# Autodesk Inventor assembly: Upperarm
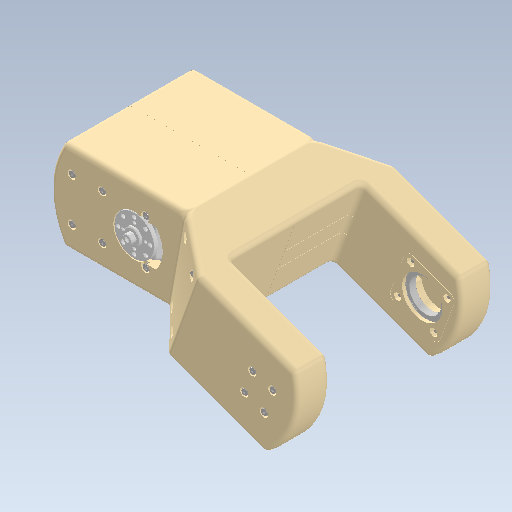
[picture p0: Inventor's stored thumbnail of the model, 512x512]
Saved by Autodesk Inventor 2021 (Build 250183000, 183)
## iProperties
Created: 2020-02-11
Part Number: Upperarm
Document SubType Name: Assembly
Designer: JochenAlt
Author: JochenAlt
## Documents named in this file (7)
- C:\Users\Jochen Alt\Documents\Daten\Projects\MiniBot\CAD\Upperarm.iam
- C:\Users\Jochen Alt\Documents\Daten\Projects\MiniBot\CAD\Upperarm.ipt
- C:\Users\Jochen Alt\Documents\Daten\Projects\MiniBot\CAD\extern\Herkulex\Herkulex DRS-040x.ipt
- C:\Users\Jochen Alt\Documents\Daten\Projects\MiniBot\CAD\extern\bearings\20x27x4\W 61704-2ZS.iam
- D:\Projects\MiniBot\CAD\extern\DIN 912\DIN 912 - M2 x 0,4 x 20 x 19.ipt
- D:\Projects\MiniBot\CAD\extern\DIN 912\DIN 912 - M2 x 0.4 x 10 x 9.ipt
- D:\Projects\MiniBot\CAD\extern\DIN 912\DIN 912 - M2 x 0,4 x 16 x 15.ipt
## Components (32 placed, 6 different names)
1. Upperarm:1 — Winkel:1, Passend:3, Fluchtend:2, Insert:1, Insert:2, Insert:3, Insert:4, Insert:5, Insert:6, Insert:7, Insert:8, Insert:9, Insert:10, Insert:11, Insert:12, Insert:13, Insert:14, Insert:15, Insert:16, Insert:17, Insert:18, Insert:19, Insert:20, Insert:21, Insert:22, Insert:23, Insert:24, Insert:25, Insert:26, Insert:27, Insert:28, Mate:4, Mate:5
2. Herkulex DRS-040x:1 — Passend:1, Passend:2, Fluchtend:1, Winkel:1
3. Herkulex DRS-040x:2 — Passend:1, Passend:2, Fluchtend:1, Passend:3, Fluchtend:2
4. DIN 912 - replaced by DIN EN ISO 4762 M2 x 20:1 — Insert:1
5. DIN 912 - replaced by DIN EN ISO 4762 M2 x 20:2 — Insert:2
6. DIN 912 - replaced by DIN EN ISO 4762 M2 x 20:3 — Insert:3
7. DIN 912 - replaced by DIN EN ISO 4762 M2 x 20:4 — Insert:4
8. DIN 912 - replaced by DIN EN ISO 4762 M2 x 10:1 — Insert:5
9. DIN 912 - replaced by DIN EN ISO 4762 M2 x 10:2 — Insert:6
10. DIN 912 - replaced by DIN EN ISO 4762 M2 x 10:3 — Insert:7
11. DIN 912 - replaced by DIN EN ISO 4762 M2 x 10:4 — Insert:8
12. DIN 912 - replaced by DIN EN ISO 4762 M2 x 10:5 — Insert:9
13. DIN 912 - replaced by DIN EN ISO 4762 M2 x 10:6 — Insert:10
14. DIN 912 - replaced by DIN EN ISO 4762 M2 x 10:7 — Insert:11
15. DIN 912 - replaced by DIN EN ISO 4762 M2 x 10:8 — Insert:12
16. DIN 912 - replaced by DIN EN ISO 4762 M2 x 10:9 — Insert:13
17. DIN 912 - replaced by DIN EN ISO 4762 M2 x 10:10 — Insert:14
18. DIN 912 - replaced by DIN EN ISO 4762 M2 x 10:11 — Insert:15
19. DIN 912 - replaced by DIN EN ISO 4762 M2 x 10:12 — Insert:16
20. DIN 912 - replaced by DIN EN ISO 4762 M2 x 20:5 — Insert:17
21. DIN 912 - replaced by DIN EN ISO 4762 M2 x 20:6 — Insert:18
22. DIN 912 - replaced by DIN EN ISO 4762 M2 x 16:1 — Insert:19
23. DIN 912 - replaced by DIN EN ISO 4762 M2 x 16:2 — Insert:20
24. DIN 912 - replaced by DIN EN ISO 4762 M2 x 16:3 — Insert:21
25. DIN 912 - replaced by DIN EN ISO 4762 M2 x 16:4 — Insert:22
26. DIN 912 - replaced by DIN EN ISO 4762 M2 x 20:7 — Insert:23
27. DIN 912 - replaced by DIN EN ISO 4762 M2 x 20:8 — Insert:24
28. DIN 912 - replaced by DIN EN ISO 4762 M2 x 20:9 — Insert:25
29. DIN 912 - replaced by DIN EN ISO 4762 M2 x 20:10 — Insert:26
30. DIN 912 - replaced by DIN EN ISO 4762 M2 x 20:11 — Insert:27
31. DIN 912 - replaced by DIN EN ISO 4762 M2 x 20:12 — Insert:28
32. W 61704-2ZS:1 [sub-assembly] — Mate:4, Mate:5
## Relationships (36: Insert 28, Mate 5, Flush 2, Angle 1)
- Passend:1 [Mate]: Herkulex DRS-040x:1 ↔ Herkulex DRS-040x:2
- Passend:2 [Mate] (0.2 mm): Herkulex DRS-040x:1 ↔ Herkulex DRS-040x:2
- Fluchtend:1 [Flush]: Herkulex DRS-040x:1 ↔ Herkulex DRS-040x:2
- Winkel:1 [Angle] (-90 deg): Upperarm:1 ↔ Herkulex DRS-040x:1
- Passend:3 [Mate]: Upperarm:1 ↔ Herkulex DRS-040x:2
- Fluchtend:2 [Flush]: Upperarm:1 ↔ Herkulex DRS-040x:2
- Insert:1: Upperarm:1 ↔ DIN 912 - replaced by DIN EN ISO 4762 M2 x 20:1
- Insert:2: Upperarm:1 ↔ DIN 912 - replaced by DIN EN ISO 4762 M2 x 20:2
- Insert:3: Upperarm:1 ↔ DIN 912 - replaced by DIN EN ISO 4762 M2 x 20:3
- Insert:4: Upperarm:1 ↔ DIN 912 - replaced by DIN EN ISO 4762 M2 x 20:4
- Insert:5: Upperarm:1 ↔ DIN 912 - replaced by DIN EN ISO 4762 M2 x 10:1
- Insert:6: Upperarm:1 ↔ DIN 912 - replaced by DIN EN ISO 4762 M2 x 10:2
- Insert:7: Upperarm:1 ↔ DIN 912 - replaced by DIN EN ISO 4762 M2 x 10:3
- Insert:8: Upperarm:1 ↔ DIN 912 - replaced by DIN EN ISO 4762 M2 x 10:4
- Insert:9: Upperarm:1 ↔ DIN 912 - replaced by DIN EN ISO 4762 M2 x 10:5
- Insert:10: Upperarm:1 ↔ DIN 912 - replaced by DIN EN ISO 4762 M2 x 10:6
- Insert:11: Upperarm:1 ↔ DIN 912 - replaced by DIN EN ISO 4762 M2 x 10:7
- Insert:12: Upperarm:1 ↔ DIN 912 - replaced by DIN EN ISO 4762 M2 x 10:8
- Insert:13: Upperarm:1 ↔ DIN 912 - replaced by DIN EN ISO 4762 M2 x 10:9
- Insert:14: Upperarm:1 ↔ DIN 912 - replaced by DIN EN ISO 4762 M2 x 10:10
- Insert:15: Upperarm:1 ↔ DIN 912 - replaced by DIN EN ISO 4762 M2 x 10:11
- Insert:16: Upperarm:1 ↔ DIN 912 - replaced by DIN EN ISO 4762 M2 x 10:12
- Insert:17: Upperarm:1 ↔ DIN 912 - replaced by DIN EN ISO 4762 M2 x 20:5
- Insert:18: Upperarm:1 ↔ DIN 912 - replaced by DIN EN ISO 4762 M2 x 20:6
- Insert:19: Upperarm:1 ↔ DIN 912 - replaced by DIN EN ISO 4762 M2 x 16:1
- Insert:20: Upperarm:1 ↔ DIN 912 - replaced by DIN EN ISO 4762 M2 x 16:2
- Insert:21: Upperarm:1 ↔ DIN 912 - replaced by DIN EN ISO 4762 M2 x 16:3
- Insert:22: Upperarm:1 ↔ DIN 912 - replaced by DIN EN ISO 4762 M2 x 16:4
- Insert:23: Upperarm:1 ↔ DIN 912 - replaced by DIN EN ISO 4762 M2 x 20:7
- Insert:24: Upperarm:1 ↔ DIN 912 - replaced by DIN EN ISO 4762 M2 x 20:8
- Insert:25: Upperarm:1 ↔ DIN 912 - replaced by DIN EN ISO 4762 M2 x 20:9
- Insert:26: Upperarm:1 ↔ DIN 912 - replaced by DIN EN ISO 4762 M2 x 20:10
- Insert:27: Upperarm:1 ↔ DIN 912 - replaced by DIN EN ISO 4762 M2 x 20:11
- Insert:28: Upperarm:1 ↔ DIN 912 - replaced by DIN EN ISO 4762 M2 x 20:12
- Mate:4: Upperarm:1 ↔ W 61704-2ZS:1
- Mate:5: Upperarm:1 ↔ W 61704-2ZS:1
